# Autodesk Inventor assembly: Quadropod_assemblie
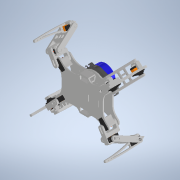
[picture p0: Inventor's stored thumbnail of the model, 180x180]
Saved by Autodesk Inventor 2020.3 (Build 243373000, 373)
## iProperties
Created: 2021-03-19
Part Number: Quadropod_assemblie
Document SubType Name: Assembly
Designer: sanyi
Author: sanyi
## Documents named in this file (9)
- C:\Users\sanyi\OneDrive\Dokumentumok\Inventor\Quadropod\Quadropod_assemblie.iam
- C:\Users\sanyi\OneDrive\Dokumentumok\Inventor\Quadropod\BaseTop_v1.ipt
- C:\Users\sanyi\OneDrive\Dokumentumok\Inventor\Quadropod\ydlidar x4.ipt
- C:\Users\sanyi\OneDrive\Dokumentumok\Inventor\Quadropod\LegPin_Side_v1.ipt
- C:\Users\sanyi\OneDrive\Dokumentumok\Inventor\Quadropod\BaseBottom_v1.ipt
- C:\Users\sanyi\OneDrive\Dokumentumok\Inventor\Quadropod\LegPin_Side_v1_MIR.ipt
- C:\Users\sanyi\OneDrive\Dokumentumok\Inventor\Quadropod\LegPin_Middle_v1.ipt
- C:\Users\sanyi\OneDrive\Dokumentumok\Inventor\Quadropod\Leg_Right_v1.iam
- C:\Users\sanyi\OneDrive\Dokumentumok\Inventor\Quadropod\Leg_Right_v1_MIR.iam
## Components (13 placed, 8 different names)
1. BaseTop_v1:1 — Mate:1, Mate:2, Mate:3, Insert:13, Insert:14
2. ydlidar x4:1 — Mate:1, Mate:2, Mate:3, Flush:2
3. LegPin_Side_v1:1 — Insert:1, Insert:2
4. BaseBottom_v1:1 — Mate:4, Mate:5, Mate:6, Insert:1, Insert:2, Insert:3, Insert:4, Insert:5, Insert:6, Insert:7, Insert:8, Insert:9, Insert:10, Insert:11, Insert:12, Mate:7, Insert:15, Angle:1, Insert:16, Angle:2, Insert:17, Insert:18, Angle:3, Angle:4
5. LegPin_Side_v1_MIR:1 — Insert:11, Insert:12
6. LegPin_Middle_v1:1 — Insert:3, Insert:4, Insert:13
7. LegPin_Middle_v1:2 — Insert:5, Insert:6
8. LegPin_Middle_v1:3 — Insert:7, Insert:8, Insert:14
9. LegPin_Middle_v1:4 — Insert:9, Insert:10
10. Leg_Right_v1:1 [sub-assembly] — Mate:7, Insert:15, Angle:1
11. Leg_Right_v1:2 [sub-assembly] — Insert:16, Angle:2
12. Leg_Right_v1_MIR:1 [sub-assembly] — Insert:17, Angle:3
13. Leg_Right_v1_MIR:2 [sub-assembly] — Insert:18, Angle:4
## Relationships (31: Insert 18, Mate 7, Angle 4, Flush 2)
- Mate:1: BaseTop_v1:1 ↔ ydlidar x4:1
- Mate:2: BaseTop_v1:1 ↔ ydlidar x4:1
- Mate:3: BaseTop_v1:1 ↔ ydlidar x4:1
- Mate:4: BaseBottom_v1:1
- Flush:1 (45 mm)
- Mate:5: BaseBottom_v1:1
- Mate:6: BaseBottom_v1:1
- Insert:1: LegPin_Side_v1:1 ↔ BaseBottom_v1:1
- Insert:2: LegPin_Side_v1:1 ↔ BaseBottom_v1:1
- Insert:3: BaseBottom_v1:1 ↔ LegPin_Middle_v1:1
- Insert:4: BaseBottom_v1:1 ↔ LegPin_Middle_v1:1
- Insert:5: BaseBottom_v1:1 ↔ LegPin_Middle_v1:2
- Insert:6: BaseBottom_v1:1 ↔ LegPin_Middle_v1:2
- Insert:7: BaseBottom_v1:1 ↔ LegPin_Middle_v1:3
- Insert:8: BaseBottom_v1:1 ↔ LegPin_Middle_v1:3
- Insert:9: BaseBottom_v1:1 ↔ LegPin_Middle_v1:4
- Insert:10: BaseBottom_v1:1 ↔ LegPin_Middle_v1:4
- Insert:11: BaseBottom_v1:1 ↔ LegPin_Side_v1_MIR:1
- Insert:12: BaseBottom_v1:1 ↔ LegPin_Side_v1_MIR:1
- Insert:13: BaseTop_v1:1 ↔ LegPin_Middle_v1:1
- Insert:14: BaseTop_v1:1 ↔ LegPin_Middle_v1:3
- Mate:7: BaseBottom_v1:1 ↔ Leg_Right_v1:1
- Insert:15: BaseBottom_v1:1 ↔ Leg_Right_v1:1
- Angle:1 (180 deg): BaseBottom_v1:1 ↔ Leg_Right_v1:1
- Insert:16: BaseBottom_v1:1 ↔ Leg_Right_v1:2
- Angle:2 (180 deg): BaseBottom_v1:1 ↔ Leg_Right_v1:2
- Insert:17: BaseBottom_v1:1 ↔ Leg_Right_v1_MIR:1
- Insert:18: BaseBottom_v1:1 ↔ Leg_Right_v1_MIR:2
- Angle:3 (180 deg): BaseBottom_v1:1 ↔ Leg_Right_v1_MIR:1
- Angle:4 (0 deg): BaseBottom_v1:1 ↔ Leg_Right_v1_MIR:2
- Flush:2 (-9.4 mm): ydlidar x4:1
